# Autodesk Inventor assembly: 8100_Tx_Filter_Stage2_Layout_v1
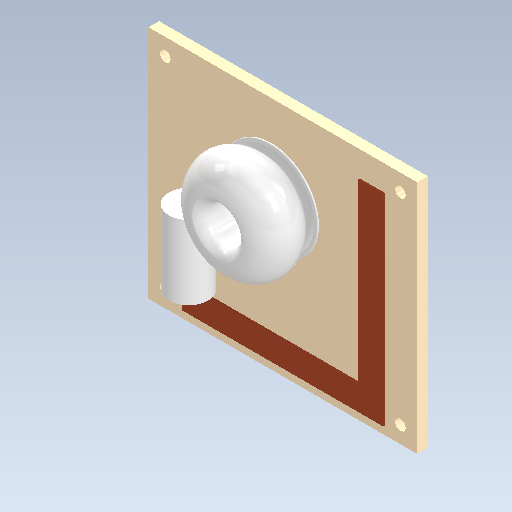
[picture p0: Inventor's stored thumbnail of the model, 512x512]
Saved by Autodesk Inventor 2021 (Build 250183000, 183)
## iProperties
Created: 2021-04-07
Part Number: 8100_Tx_Filter_Stage2_Layout_v1
Document SubType Name: Assembly
Designer: Barksdale
Author: Barksdale
## Documents named in this file (6)
- C:\Users\Barksdale\Dropbox (MIT)\MPI Group Folder\MPS\Inventor_Parts and MPSv2 all folder\MPSV2\Tx Filter\8100_Tx_Filter_Stage2_Layout_v1.iam
- C:\Users\Barksdale\Dropbox (MIT)\MPI Group Folder\MPS\Inventor_Parts and MPSv2 all folder\MPSV2\Tx Filter\8020_Base_Tx_Filter_v1.ipt
- C:\Users\Barksdale\Dropbox (MIT)\MPI Group Folder\MPS\Inventor_Parts and MPSv2 all folder\MPSV2\Tx Filter\8004_65uH_DCore_2layer_Tx_Filter_MPSv2_v1.ipt
- C:\Users\Barksdale\Dropbox (MIT)\MPI Group Folder\MPS\Inventor_Parts and MPSv2 all folder\MPSV2\Tx Filter\8002_base_132uH_DCore_2layer_Tx_Filter_MPSv2_v1.ipt
- C:\Users\Barksdale\Dropbox (MIT)\MPI Group Folder\MPS\Inventor_Parts and MPSv2 all folder\MPSV2\Tx Filter\8011_1uF_Tx_Capacitor_v1.ipt
- C:\Users\Barksdale\Dropbox (MIT)\MPI Group Folder\MPS\Inventor_Parts and MPSv2 all folder\MPSV2\Tx Filter\8006_Cu_groundplane_Tx_Filter_Stage2_MPSv2_v1.ipt
## Components (5 placed, 5 different names)
1. 8020_Base_Tx_Filter_v1:1 — Tangent:1, Mate:1, Mate:4, Flush:1
2. 8004_65uH_DCore_2layer_Tx_Filter_MPSv2_v1:1 — Mate:2, Mate:3
3. 8002_base_132uH_DCore_2layer_Tx_Filter_MPSv2_v1:1 — Mate:1, Mate:2, Mate:3
4. 8011_1uF_Tx_Capacitor_v1:1 — Tangent:1
5. 8006_Cu_groundplane_Tx_Filter_Stage2_MPSv2_v1:1 — Mate:4, Flush:1
## Relationships (6: Mate 4, Tangent 1, Flush 1)
- Tangent:1: 8020_Base_Tx_Filter_v1:1 ↔ 8011_1uF_Tx_Capacitor_v1:1
- Mate:1: 8020_Base_Tx_Filter_v1:1 ↔ 8002_base_132uH_DCore_2layer_Tx_Filter_MPSv2_v1:1
- Mate:2: 8004_65uH_DCore_2layer_Tx_Filter_MPSv2_v1:1 ↔ 8002_base_132uH_DCore_2layer_Tx_Filter_MPSv2_v1:1
- Mate:3: 8004_65uH_DCore_2layer_Tx_Filter_MPSv2_v1:1 ↔ 8002_base_132uH_DCore_2layer_Tx_Filter_MPSv2_v1:1
- Mate:4: 8020_Base_Tx_Filter_v1:1 ↔ 8006_Cu_groundplane_Tx_Filter_Stage2_MPSv2_v1:1
- Flush:1 (5 mm): 8020_Base_Tx_Filter_v1:1 ↔ 8006_Cu_groundplane_Tx_Filter_Stage2_MPSv2_v1:1
